# Autodesk Inventor assembly: Tail
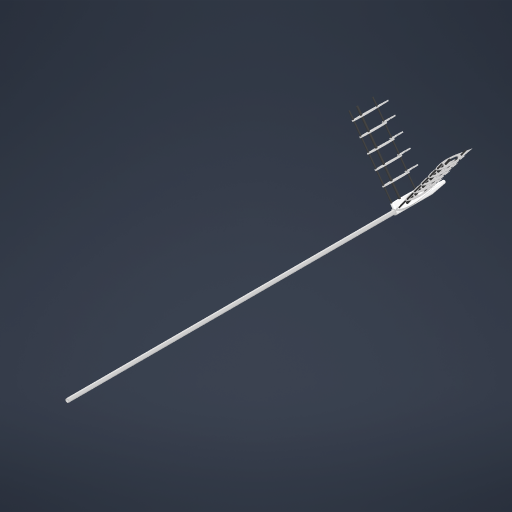
[picture p0: Inventor's stored thumbnail of the model, 512x512]
Saved by Autodesk Inventor 2023 (Build 270158000, 158)
## iProperties
Created: 2023-01-05
Part Number: Tail
Document SubType Name: Assembly
Designer: szykr
Author: szykr
## Documents named in this file (7)
- D:\Folder Instalacyjny\GitHub Pliki\Solaris\new model\Tail\Tail.iam
- D:\Folder Instalacyjny\GitHub Pliki\Solaris\new model\wingspar.ipt
- D:\Folder Instalacyjny\GitHub Pliki\Solaris\new model\Tail\Tmount.ipt
- D:\Folder Instalacyjny\GitHub Pliki\Solaris\new model\Tail\Tżebro default.ipt
- D:\Folder Instalacyjny\GitHub Pliki\Solaris\new model\Tail\Twingspar.ipt
- D:\Folder Instalacyjny\GitHub Pliki\Solaris\new model\Tail\TsmallSpar.ipt
- D:\Folder Instalacyjny\GitHub Pliki\Solaris\new model\Tail\Zebro_z_lotka.iam
## Components (20 placed, 6 different names)
1. wingspar:1 — Insert:1
2. Tmount:1 — Insert:1, Insert:2, Insert:3, Insert:4, Insert:5, Insert:6, Insert:10, Insert:14, Insert:15, Insert:16, Insert:17
3. Tżebro default:1 — Insert:4, Insert:5
4. Tżebro default:2 — Insert:2, Insert:3, Insert:7, Insert:12, Insert:13
5. Twingspar:1 — Insert:7
6. Twingspar:2 — Insert:6
7. TsmallSpar:1 — Insert:10
8. TsmallSpar:2 — Mate:2, Mate:3
9. TsmallSpar:3 — Insert:12
10. TsmallSpar:4 — Insert:13, Mate:1, Mate:4
11. Tżebro default:3 — Insert:16, Mate:3
12. Tżebro default:4 — Insert:17, Mate:4
13. Zebro_z_lotka:1 [sub-assembly] — Insert:14, Mate:1
14. Zebro_z_lotka:3 [sub-assembly]
15. Zebro_z_lotka:4 [sub-assembly]
16. Zebro_z_lotka:5 [sub-assembly]
17. Zebro_z_lotka:2 [sub-assembly] — Insert:15, Mate:2
18. Zebro_z_lotka:6 [sub-assembly]
19. Zebro_z_lotka:7 [sub-assembly]
20. Zebro_z_lotka:8 [sub-assembly]
## Component patterns: (4 elements, first: Zebro_z_lotka:1), (4 elements, first: Zebro_z_lotka:2)
## Relationships (18: Insert 14, Mate 4)
- Insert:1: wingspar:1 ↔ Tmount:1
- Insert:2: Tmount:1 ↔ Tżebro default:2
- Insert:3: Tmount:1 ↔ Tżebro default:2
- Insert:4: Tmount:1 ↔ Tżebro default:1
- Insert:5: Tmount:1 ↔ Tżebro default:1
- Insert:6 (-10 mm): Tmount:1 ↔ Twingspar:2
- Insert:7 (-10 mm): Tżebro default:2 ↔ Twingspar:1
- Insert:10 (-9.633 mm): Tmount:1 ↔ TsmallSpar:1
- Insert:12 (-9.633 mm): Tżebro default:2 ↔ TsmallSpar:3
- Insert:13 (-9.633 mm): Tżebro default:2 ↔ TsmallSpar:4
- Insert:14 (35.5 mm): Tmount:1 ↔ Zebro_z_lotka:1
- Mate:1: TsmallSpar:4 ↔ Zebro_z_lotka:1
- Insert:15 (35.5 mm): Tmount:1 ↔ Zebro_z_lotka:2
- Mate:2: TsmallSpar:2 ↔ Zebro_z_lotka:2
- Insert:16 (177.5 mm): Tmount:1 ↔ Tżebro default:3
- Mate:3: TsmallSpar:2 ↔ Tżebro default:3
- Insert:17 (177.5 mm): Tmount:1 ↔ Tżebro default:4
- Mate:4: TsmallSpar:4 ↔ Tżebro default:4
## Named parameters: dlugosc = 213 mm, lotki = 4, ilosc_zeber = 6, spacing = 35.5 mm
